# Autodesk Inventor assembly: Reflow Oven Assembly
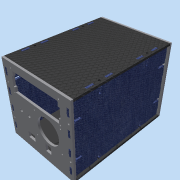
[picture p0: Inventor's stored thumbnail of the model, 180x180]
Saved by Autodesk Inventor 2013 (Build 170138000, 138)
## iProperties
Created: 2012-12-29
Part Number: Reflow Oven Assembly
Document SubType Name: Assembly
Designer: Administrator
Author: Administrator
## Documents named in this file (6)
- Z:\Dropbox\Projects\Reflow Oven\Box\Reflow Oven Assembly.iam
- Z:\Dropbox\Projects\Reflow Oven\Box\Box Front.ipt
- Z:\Dropbox\Projects\Reflow Oven\Box\Box Back.ipt
- Z:\Dropbox\Projects\Reflow Oven\Box\Box Side Panel.ipt
- Z:\Dropbox\Projects\Reflow Oven\Box\Box Top.ipt
- Z:\Dropbox\Projects\Reflow Oven\Box\Box Bottom.ipt
## Components (6 placed, 5 different names)
1. Box Front:1 — Mate:2, Flush:2, Mate:4, Mate:5, Mate:6, Mate:7
2. Box Back:1 — Mate:1, Flush:1, Flush:3, Flush:4, Mate:3
3. Box Side Panel:1 — Mate:5, Mate:6
4. Box Side Panel:2 — Mate:3, Mate:4, Mate:7
5. Box Top:1 — Mate:1, Flush:1, Mate:2, Flush:2
6. Box Bottom:1 — Flush:3, Flush:4
## Relationships (11: Mate 7, Flush 4)
- Mate:1: Box Back:1 ↔ Box Top:1
- Flush:1: Box Back:1 ↔ Box Top:1
- Mate:2: Box Front:1 ↔ Box Top:1
- Flush:2: Box Front:1 ↔ Box Top:1
- Flush:3: Box Back:1 ↔ Box Bottom:1
- Flush:4: Box Back:1 ↔ Box Bottom:1
- Mate:3: Box Back:1 ↔ Box Side Panel:2
- Mate:4: Box Front:1 ↔ Box Side Panel:2
- Mate:5: Box Front:1 ↔ Box Side Panel:1
- Mate:6: Box Front:1 ↔ Box Side Panel:1
- Mate:7: Box Front:1 ↔ Box Side Panel:2
